# Autodesk Inventor assembly: Mini - 360
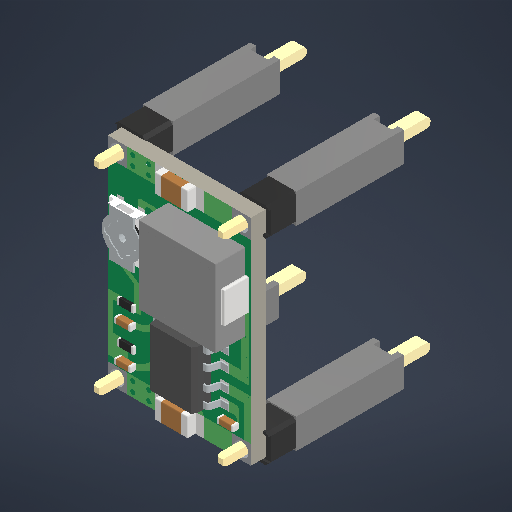
[picture p0: Inventor's stored thumbnail of the model, 512x512]
Saved by Autodesk Inventor 2026.1 (Build 301233020, 233B)
## iProperties
Created: 2026-02-14
Part Number: Mini - 360
Document SubType Name: Assembly
Designer: celio
Author: celio
## Documents named in this file (4)
- C:\Users\celio\OneDrive\Documentos\Inventor\ZeGuia\Componentes\Regulador\Mini - 360.iam
- C:\Users\celio\OneDrive\Documentos\Inventor\ZeGuia\Componentes\Regulador\MIni - 360\MIni - 360.ipt
- C:\Users\celio\OneDrive\Documentos\Inventor\ZeGuia\Pinos\Macho\1x1\1x1.iam
- C:\Users\celio\OneDrive\Documentos\Inventor\ZeGuia\Pinos\Femea\1x1\1x1.ipt
## Components (9 placed, 2 different names)
1. MIni - 360:1 — Coincidente:1, Coincidente:2, Coincidente:3, Coincidente:4
2. 1x1:1 [sub-assembly] — Coincidente:1, Coincidente:5, Alinhado:1, Alinhado:2
3. 1x1:2 [sub-assembly] — Coincidente:2, Coincidente:6, Alinhado:3, Alinhado:4
4. 1x1:3 [sub-assembly] — Coincidente:4, Coincidente:7, Alinhado:5, Alinhado:6
5. 1x1:4 [sub-assembly] — Coincidente:3, Coincidente:8, Alinhado:7, Alinhado:8
6. 1x1:5 — Coincidente:6, Alinhado:3, Alinhado:4
7. 1x1:6 — Coincidente:7, Alinhado:5, Alinhado:6
8. 1x1:7 — Coincidente:5, Alinhado:1, Alinhado:2
9. 1x1:8 — Coincidente:8, Alinhado:7, Alinhado:8
## Relationships (16: Mate 8, Flush 8)
- Coincidente:1 [Mate]: MIni - 360:1 ↔ 1x1:1
- Coincidente:2 [Mate]: MIni - 360:1 ↔ 1x1:2
- Coincidente:3 [Mate]: MIni - 360:1 ↔ 1x1:4
- Coincidente:4 [Mate]: MIni - 360:1 ↔ 1x1:3
- Coincidente:5 [Mate]: 1x1:1 ↔ 1x1:7
- Alinhado:1 [Flush]: 1x1:1 ↔ 1x1:7
- Alinhado:2 [Flush]: 1x1:1 ↔ 1x1:7
- Coincidente:6 [Mate]: 1x1:2 ↔ 1x1:5
- Alinhado:3 [Flush]: 1x1:2 ↔ 1x1:5
- Alinhado:4 [Flush]: 1x1:2 ↔ 1x1:5
- Coincidente:7 [Mate]: 1x1:3 ↔ 1x1:6
- Alinhado:5 [Flush]: 1x1:3 ↔ 1x1:6
- Alinhado:6 [Flush]: 1x1:3 ↔ 1x1:6
- Coincidente:8 [Mate]: 1x1:4 ↔ 1x1:8
- Alinhado:7 [Flush]: 1x1:4 ↔ 1x1:8
- Alinhado:8 [Flush]: 1x1:4 ↔ 1x1:8
